# Autodesk Inventor assembly: MaleHeader
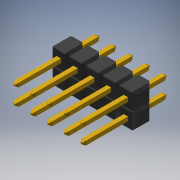
[picture p0: Inventor's stored thumbnail of the model, 180x180]
Saved by Autodesk Inventor 2018 (Build 220112000, 112)
## iProperties
Created: 2017-04-09
Part Number: MaleHeader
Document SubType Name: Assembly
Designer: dkt01
Author: dkt01
## Documents named in this file (2)
- C:\Users\dktur\Dropbox\StackLightMonitor\CAD\MaleHeader.iam
- C:\Users\dktur\Dropbox\StackLightMonitor\CAD\MaleHeader.ipt
## Components (10 placed, 1 different names)
1. MaleHeader:1
2. MaleHeader:2
3. MaleHeader:3
4. MaleHeader:4
5. MaleHeader:5
6. MaleHeader:6
7. MaleHeader:7
8. MaleHeader:8
9. MaleHeader:9
10. MaleHeader:10
## Component patterns: (10 elements, first: MaleHeader:1)
